# Autodesk Inventor assembly: Rear Hex Hub
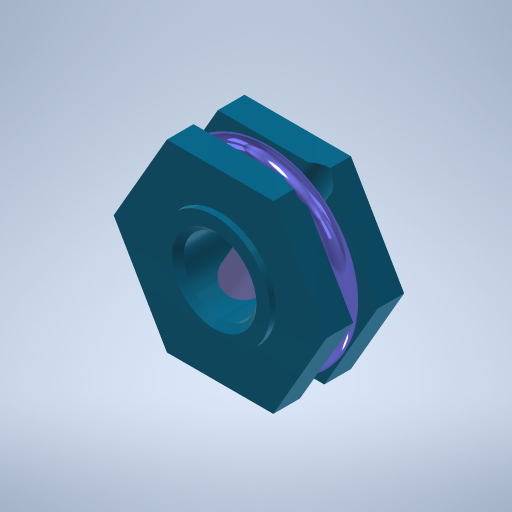
[picture p0: Inventor's stored thumbnail of the model, 512x512]
Saved by Autodesk Inventor 2023.1 (Build 271208000, 208)
## iProperties
Created: 2019-12-03
Part Number: Rear Hex Hub
Document SubType Name: Assembly
Designer: Jopa
Author: Jopa
## Documents named in this file (4)
- C:\Users\Arzum Naz Doğaner\OneDrive\Masaüstü\HUDSON süspansiyon\Rear Hex Hub.iam
- C:\Users\Arzum Naz Doğaner\OneDrive\Masaüstü\HUDSON süspansiyon\Hex Drive.ipt
- C:\Users\Arzum Naz Doğaner\OneDrive\Masaüstü\HUDSON süspansiyon\Hex Axle Pin.ipt
- C:\Users\Arzum Naz Doğaner\OneDrive\Masaüstü\HUDSON süspansiyon\Hex Retaining O-Ring.ipt
## Components (3 placed, 3 different names)
1. Hex Drive:1 — Mate:1, Mate:2, Mate:3, Mate:4
2. Hex Axle Pin:1 — Mate:1, Mate:2
3. Hex Retaining O-Ring:1 — Mate:3, Mate:4
## Relationships (4: Mate 4)
- Mate:1: Hex Drive:1 ↔ Hex Axle Pin:1
- Mate:2: Hex Drive:1 ↔ Hex Axle Pin:1
- Mate:3: Hex Drive:1 ↔ Hex Retaining O-Ring:1
- Mate:4: Hex Drive:1 ↔ Hex Retaining O-Ring:1
